# Autodesk Inventor assembly: Zusammenbau
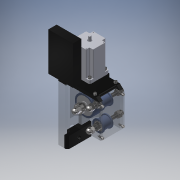
[picture p0: Inventor's stored thumbnail of the model, 180x180]
Saved by Autodesk Inventor 2019 (Build 230136000, 136)
## iProperties
Created: 2021-11-05
Part Number: Zusammenbau
Material: Generisch
Document SubType Name: Assembly
Designer: Bergi
Author: Bergi
## Documents named in this file (26)
- C:\Users\Bergi\Desktop\3D Sketches\Jalousie_Motor\Zusammenbau.iam
- C:\Users\Bergi\Desktop\3D Sketches\Jalousie_Motor\Nema23(SY60STH86-3008).ipt
- C:\Users\Bergi\Desktop\3D Sketches\Jalousie_Motor\Schneckenrad.ipt
- C:\Users\Bergi\Desktop\3D Sketches\Jalousie_Motor\Schneckenwelle.ipt
- C:\Users\Bergi\Desktop\3D Sketches\Jalousie_Motor\Gummiwalze.ipt
- C:\Users\Bergi\Desktop\3D Sketches\Jalousie_Motor\ABS Walze.ipt
- C:\Users\Bergi\Desktop\3D Sketches\Jalousie_Motor\DIN 625 T1 - 6000 - 10 x 26 x 8.ipt
- C:\Users\Bergi\Desktop\3D Sketches\Jalousie_Motor\Gewindestange.ipt
- C:\Users\Bergi\Desktop\3D Sketches\Jalousie_Motor\DIN 934 - M10 x 1,5.ipt
- C:\Users\Bergi\Desktop\3D Sketches\Jalousie_Motor\DIN 988 - 10 x 16 x 1.ipt
- C:\Users\Bergi\Desktop\3D Sketches\Jalousie_Motor\Frame.ipt
- C:\Users\Bergi\Desktop\3D Sketches\Jalousie_Motor\DIN 1587 - M10 x 1,25.ipt
- C:\Users\Bergi\Desktop\3D Sketches\Jalousie_Motor\Shaft Kupplung.ipt
- C:\Users\Bergi\Desktop\3D Sketches\Jalousie_Motor\Deckel_Frame.ipt
- C:\Users\Bergi\Desktop\3D Sketches\Jalousie_Motor\DIN 625 T1 - 626 - 6 x 19 x 6.ipt
- C:\Users\Bergi\Desktop\3D Sketches\Jalousie_Motor\Holding_Plate_Frame.ipt
- C:\Users\Bergi\Desktop\3D Sketches\Jalousie_Motor\Deckel_2_Frame.ipt
- C:\Users\Bergi\Desktop\3D Sketches\Jalousie_Motor\DIN 912 - M4 x 0,7 x 10 x 8,25.ipt
- C:\Users\Bergi\Desktop\3D Sketches\Jalousie_Motor\DIN 912 - M5 x 0,8 x 16 x 14.ipt
- C:\Users\Bergi\Desktop\3D Sketches\Jalousie_Motor\Stepperdriver.ipt
- C:\Users\Bergi\Desktop\3D Sketches\Jalousie_Motor\Zusammenbau\AIP\FEA\ds3uq4s4g.fins
- C:\Users\Bergi\Desktop\3D Sketches\Jalousie_Motor\Zusammenbau\AIP\FEA\ds3uq4s4g.fsat
- C:\Users\Bergi\Desktop\3D Sketches\Jalousie_Motor\Zusammenbau\AIP\FEA\ds3uq4s4g.ftes
- C:\Users\Bergi\Desktop\3D Sketches\Jalousie_Motor\Zusammenbau\AIP\FEA\ds3uq4s5c.fwiz
- C:\Users\Bergi\Desktop\3D Sketches\Jalousie_Motor\Zusammenbau\AIP\FEA\ds3uq4sdc.fmsh
- C:\Users\Bergi\Desktop\3D Sketches\Jalousie_Motor\Zusammenbau\AIP\FEA\ds3uq4sdd.fres
## Components (51 placed, 19 different names)
1. Nema23(SY60STH86-3008):1 — Passend:1, Winkel:1, Winkel:3, Passend:68, Winkel:4, Passend:69, Passend:71, Passend:92, Passend:93, Passend:94, Passend:95, Passend:96, Passend:97, Passend:98, Passend:99, Fluchtend:8
2. Schneckenrad:1 — Passend:2, Passend:3, Winkel:1, Passend:4, Passend:13, Passend:18
3. Schneckenwelle:1 — Passend:1, Passend:2, Passend:3
4. Gummiwalze:1 — Passend:4, Passend:13, Passend:14, Passend:16, Fluchtend:1, Passend:31
5. ABS Walze:1 — Passend:5, Passend:6, Passend:7, Passend:8, Fluchtend:1
6. DIN 625 - T1 6000 - 10 x 26 x 8:1 — Passend:6, Passend:7, Passend:36
7. DIN 625 - T1 6000 - 10 x 26 x 8:2 — Passend:5, Passend:8, Winkel:2, Passend:32, Passend:34
8. ABS Walze:2 — Passend:31
9. DIN 625 - T1 6000 - 10 x 26 x 8:3 — Passend:37, Passend:41
10. DIN 625 - T1 6000 - 10 x 26 x 8:4 — Passend:40
11. Gewindestange:1 — Passend:14, Passend:15, Passend:17, Passend:19, Passend:21, Passend:23, Passend:25, Winkel:2, Fluchtend:2, Fluchtend:3, Passend:52, Passend:54
12. DIN 934 - ersetzt durch DIN EN 24032/28673/28674 M10:1 — Passend:19, Passend:20, Passend:22
13. DIN 988 10 x 16 x 1:1 — Passend:15, Passend:16, Passend:24
14. DIN 988 10 x 16 x 1:2 — Passend:17, Passend:18, Passend:20
15. DIN 625 - T1 6000 - 10 x 26 x 8:5 — Passend:21, Passend:22, Passend:55
16. DIN 934 - ersetzt durch DIN EN 24032/28673/28674 M10:2 — Passend:23, Passend:24, Passend:26
17. DIN 625 - T1 6000 - 10 x 26 x 8:6 — Passend:25, Passend:26, Passend:42, Passend:43, Passend:53
18. Gewindestange:2 — Passend:32, Passend:33, Passend:35, Fluchtend:2, Passend:44, Passend:47, Passend:50, Passend:56, Passend:58
19. DIN 934 - ersetzt durch DIN EN 24032/28673/28674 M10:5 — Passend:33, Passend:34
20. DIN 934 - ersetzt durch DIN EN 24032/28673/28674 M10:6 — Passend:35, Passend:36
21. Gewindestange:3 — Passend:37, Passend:38, Passend:39, Fluchtend:3, Passend:45, Fluchtend:4, Passend:60, Passend:62, Passend:64, Passend:66
22. DIN 934 - ersetzt durch DIN EN 24032/28673/28674 M10:7 — Passend:38, Passend:41
23. DIN 934 - ersetzt durch DIN EN 24032/28673/28674 M10:8 — Passend:39, Passend:40
24. Frame:1 — Passend:42, Passend:43, Winkel:3, Passend:44, Passend:45, Passend:48, Passend:51, Fluchtend:4, Passend:61, Passend:63, Passend:70, Fluchtend:5, Fluchtend:6, Passend:72, Passend:73, Passend:74, Passend:75, Fluchtend:7, Passend:77, Passend:78, Passend:79
25. DIN 988 10 x 16 x 1:3 — Passend:47, Passend:48, Passend:57
26. DIN 988 10 x 16 x 1:4 — Passend:50, Passend:51, Passend:59
27. DIN 1587 M10 x 1,25 - SW16:1 — Passend:52, Passend:53
28. DIN 1587 M10 x 1,25 - SW16:2 — Passend:54, Passend:55
29. DIN 1587 M10 x 1,25 - SW16:3 — Passend:56, Passend:57
30. DIN 1587 M10 x 1,25 - SW16:4 — Passend:58, Passend:59
31. DIN 988 10 x 16 x 1:5 — Passend:60, Passend:61, Passend:67
32. DIN 988 10 x 16 x 1:6 — Passend:62, Passend:63, Passend:65
33. DIN 1587 M10 x 1,25 - SW16:5 — Passend:64, Passend:65
34. DIN 1587 M10 x 1,25 - SW16:6 — Passend:66, Passend:67
35. Shaft Kupplung:1 — Passend:68, Winkel:4, Passend:69, Passend:76
36. Deckel_Frame:1 — Passend:70, Fluchtend:5, Fluchtend:6, Passend:71, Passend:76, Passend:88, Passend:89, Passend:90, Passend:91, Passend:100, Passend:101
37. DIN 625 - T1 626 - 6 x 19 x 6:1 — Passend:72, Passend:73
38. Holding_Plate_Frame:1 — Passend:74, Passend:75, Fluchtend:7
39. Deckel_2_Frame:1 — Passend:77, Passend:78, Passend:79, Passend:80, Passend:81, Passend:82, Passend:83, Passend:84, Passend:85, Passend:86, Passend:87
40. DIN 912 - ersetzt durch DIN EN ISO 4762 M4 x 10:1 — Passend:80, Passend:81
41. DIN 912 - ersetzt durch DIN EN ISO 4762 M4 x 10:2 — Passend:82, Passend:83
42. DIN 912 - ersetzt durch DIN EN ISO 4762 M4 x 10:3 — Passend:84, Passend:85
43. DIN 912 - ersetzt durch DIN EN ISO 4762 M4 x 10:4 — Passend:86, Passend:87
44. DIN 912 - ersetzt durch DIN EN ISO 4762 M5 x 16:1 — Passend:88, Passend:89
45. DIN 912 - ersetzt durch DIN EN ISO 4762 M5 x 16:2 — Passend:90, Passend:91
46. DIN 912 - ersetzt durch DIN EN ISO 4762 M5 x 16:3 — Passend:92, Passend:98
47. DIN 912 - ersetzt durch DIN EN ISO 4762 M5 x 16:4 — Passend:95, Passend:96
48. DIN 912 - ersetzt durch DIN EN ISO 4762 M5 x 16:5 — Passend:94, Passend:99
49. DIN 912 - ersetzt durch DIN EN ISO 4762 M5 x 16:6 — Passend:93, Passend:97
50. DIN 912 - ersetzt durch DIN EN ISO 4762 M5 x 16:7 — Passend:100, Passend:101
51. Stepperdriver:1 — Fluchtend:8
## Relationships (107: Mate 95, Flush 8, Angle 4)
- Passend:1 [Mate]: Nema23(SY60STH86-3008):1 ↔ Schneckenwelle:1
- Passend:2 [Mate]: Schneckenrad:1 ↔ Schneckenwelle:1
- Passend:3 [Mate] (-6.5 mm): Schneckenrad:1 ↔ Schneckenwelle:1
- Winkel:1 [Angle] (-90 deg): Nema23(SY60STH86-3008):1 ↔ Schneckenrad:1
- Passend:4 [Mate]: Schneckenrad:1 ↔ Gummiwalze:1
- Passend:5 [Mate]: ABS Walze:1 ↔ DIN 625 - T1 6000 - 10 x 26 x 8:2
- Passend:6 [Mate]: ABS Walze:1 ↔ DIN 625 - T1 6000 - 10 x 26 x 8:1
- Passend:7 [Mate]: ABS Walze:1 ↔ DIN 625 - T1 6000 - 10 x 26 x 8:1
- Passend:8 [Mate]: ABS Walze:1 ↔ DIN 625 - T1 6000 - 10 x 26 x 8:2
- [Mate]: ABS Walze:2 ↔ DIN 625 - T1 6000 - 10 x 26 x 8:4
- [Mate]: ABS Walze:2 ↔ DIN 625 - T1 6000 - 10 x 26 x 8:3
- [Mate]: ABS Walze:2 ↔ DIN 625 - T1 6000 - 10 x 26 x 8:3
- [Mate]: ABS Walze:2 ↔ DIN 625 - T1 6000 - 10 x 26 x 8:4
- Passend:13 [Mate]: Schneckenrad:1 ↔ Gummiwalze:1
- Passend:14 [Mate]: Gummiwalze:1 ↔ Gewindestange:1
- Passend:15 [Mate]: Gewindestange:1 ↔ DIN 988 10 x 16 x 1:1
- Passend:16 [Mate]: Gummiwalze:1 ↔ DIN 988 10 x 16 x 1:1
- Passend:17 [Mate]: Gewindestange:1 ↔ DIN 988 10 x 16 x 1:2
- Passend:18 [Mate]: Schneckenrad:1 ↔ DIN 988 10 x 16 x 1:2
- Passend:19 [Mate]: Gewindestange:1 ↔ DIN 934 - ersetzt durch DIN EN 24032/28673/28674 M10:1
- Passend:20 [Mate]: DIN 934 - ersetzt durch DIN EN 24032/28673/28674 M10:1 ↔ DIN 988 10 x 16 x 1:2
- Passend:21 [Mate]: Gewindestange:1 ↔ DIN 625 - T1 6000 - 10 x 26 x 8:5
- Passend:22 [Mate]: DIN 934 - ersetzt durch DIN EN 24032/28673/28674 M10:1 ↔ DIN 625 - T1 6000 - 10 x 26 x 8:5
- Passend:23 [Mate]: Gewindestange:1 ↔ DIN 934 - ersetzt durch DIN EN 24032/28673/28674 M10:2
- Passend:24 [Mate]: DIN 988 10 x 16 x 1:1 ↔ DIN 934 - ersetzt durch DIN EN 24032/28673/28674 M10:2
- Passend:25 [Mate]: Gewindestange:1 ↔ DIN 625 - T1 6000 - 10 x 26 x 8:6
- Passend:26 [Mate]: DIN 934 - ersetzt durch DIN EN 24032/28673/28674 M10:2 ↔ DIN 625 - T1 6000 - 10 x 26 x 8:6
- Winkel:2 [Angle] (0 deg): DIN 625 - T1 6000 - 10 x 26 x 8:2 ↔ Gewindestange:1
- Fluchtend:1 [Flush]: Gummiwalze:1 ↔ ABS Walze:1
- Passend:31 [Mate]: Gummiwalze:1 ↔ ABS Walze:2
- Passend:32 [Mate]: DIN 625 - T1 6000 - 10 x 26 x 8:2 ↔ Gewindestange:2
- Passend:33 [Mate]: Gewindestange:2 ↔ DIN 934 - ersetzt durch DIN EN 24032/28673/28674 M10:5
- Passend:34 [Mate]: DIN 625 - T1 6000 - 10 x 26 x 8:2 ↔ DIN 934 - ersetzt durch DIN EN 24032/28673/28674 M10:5
- Passend:35 [Mate]: Gewindestange:2 ↔ DIN 934 - ersetzt durch DIN EN 24032/28673/28674 M10:6
- Passend:36 [Mate]: DIN 625 - T1 6000 - 10 x 26 x 8:1 ↔ DIN 934 - ersetzt durch DIN EN 24032/28673/28674 M10:6
- Passend:37 [Mate]: DIN 625 - T1 6000 - 10 x 26 x 8:3 ↔ Gewindestange:3
- Passend:38 [Mate]: Gewindestange:3 ↔ DIN 934 - ersetzt durch DIN EN 24032/28673/28674 M10:7
- Passend:39 [Mate]: Gewindestange:3 ↔ DIN 934 - ersetzt durch DIN EN 24032/28673/28674 M10:8
- Passend:40 [Mate]: DIN 625 - T1 6000 - 10 x 26 x 8:4 ↔ DIN 934 - ersetzt durch DIN EN 24032/28673/28674 M10:8
- Passend:41 [Mate]: DIN 625 - T1 6000 - 10 x 26 x 8:3 ↔ DIN 934 - ersetzt durch DIN EN 24032/28673/28674 M10:7
- Fluchtend:2 [Flush]: Gewindestange:1 ↔ Gewindestange:2
- Fluchtend:3 [Flush]: Gewindestange:1 ↔ Gewindestange:3
- Passend:42 [Mate]: DIN 625 - T1 6000 - 10 x 26 x 8:6 ↔ Frame:1
- Passend:43 [Mate]: DIN 625 - T1 6000 - 10 x 26 x 8:6 ↔ Frame:1
- Winkel:3 [Angle] (0 deg): Nema23(SY60STH86-3008):1 ↔ Frame:1
- Passend:44 [Mate]: Gewindestange:2 ↔ Frame:1
- Passend:45 [Mate]: Gewindestange:3 ↔ Frame:1
- Passend:47 [Mate]: Gewindestange:2 ↔ DIN 988 10 x 16 x 1:3
- Passend:48 [Mate]: Frame:1 ↔ DIN 988 10 x 16 x 1:3
- Passend:50 [Mate]: Gewindestange:2 ↔ DIN 988 10 x 16 x 1:4
- Passend:51 [Mate]: Frame:1 ↔ DIN 988 10 x 16 x 1:4
- Passend:52 [Mate]: Gewindestange:1 ↔ DIN 1587 M10 x 1,25 - SW16:1
- Passend:53 [Mate]: DIN 625 - T1 6000 - 10 x 26 x 8:6 ↔ DIN 1587 M10 x 1,25 - SW16:1
- Passend:54 [Mate]: Gewindestange:1 ↔ DIN 1587 M10 x 1,25 - SW16:2
- Passend:55 [Mate]: DIN 625 - T1 6000 - 10 x 26 x 8:5 ↔ DIN 1587 M10 x 1,25 - SW16:2
- Passend:56 [Mate]: Gewindestange:2 ↔ DIN 1587 M10 x 1,25 - SW16:3
- Passend:57 [Mate]: DIN 988 10 x 16 x 1:3 ↔ DIN 1587 M10 x 1,25 - SW16:3
- Passend:58 [Mate]: Gewindestange:2 ↔ DIN 1587 M10 x 1,25 - SW16:4
- Passend:59 [Mate]: DIN 988 10 x 16 x 1:4 ↔ DIN 1587 M10 x 1,25 - SW16:4
- Fluchtend:4 [Flush] (8 mm): Gewindestange:3 ↔ Frame:1
- Passend:60 [Mate]: Gewindestange:3 ↔ DIN 988 10 x 16 x 1:5
- Passend:61 [Mate]: Frame:1 ↔ DIN 988 10 x 16 x 1:5
- Passend:62 [Mate]: Gewindestange:3 ↔ DIN 988 10 x 16 x 1:6
- Passend:63 [Mate]: Frame:1 ↔ DIN 988 10 x 16 x 1:6
- Passend:64 [Mate]: Gewindestange:3 ↔ DIN 1587 M10 x 1,25 - SW16:5
- Passend:65 [Mate]: DIN 988 10 x 16 x 1:6 ↔ DIN 1587 M10 x 1,25 - SW16:5
- Passend:66 [Mate]: Gewindestange:3 ↔ DIN 1587 M10 x 1,25 - SW16:6
- Passend:67 [Mate]: DIN 988 10 x 16 x 1:5 ↔ DIN 1587 M10 x 1,25 - SW16:6
- Passend:68 [Mate]: Nema23(SY60STH86-3008):1 ↔ Shaft Kupplung:1
- Winkel:4 [Angle] (0 deg): Nema23(SY60STH86-3008):1 ↔ Shaft Kupplung:1
- Passend:69 [Mate] (1 mm): Nema23(SY60STH86-3008):1 ↔ Shaft Kupplung:1
- Passend:70 [Mate]: Frame:1 ↔ Deckel_Frame:1
- Fluchtend:5 [Flush]: Frame:1 ↔ Deckel_Frame:1
- Fluchtend:6 [Flush]: Frame:1 ↔ Deckel_Frame:1
- Passend:71 [Mate]: Nema23(SY60STH86-3008):1 ↔ Deckel_Frame:1
- Passend:72 [Mate]: Frame:1 ↔ DIN 625 - T1 626 - 6 x 19 x 6:1
- Passend:73 [Mate]: Frame:1 ↔ DIN 625 - T1 626 - 6 x 19 x 6:1
- Passend:74 [Mate]: Frame:1 ↔ Holding_Plate_Frame:1
- Passend:75 [Mate]: Frame:1 ↔ Holding_Plate_Frame:1
- Fluchtend:7 [Flush]: Frame:1 ↔ Holding_Plate_Frame:1
- Passend:76 [Mate]: Shaft Kupplung:1 ↔ Deckel_Frame:1
- Passend:77 [Mate]: Frame:1 ↔ Deckel_2_Frame:1
- Passend:78 [Mate]: Frame:1 ↔ Deckel_2_Frame:1
- Passend:79 [Mate]: Frame:1 ↔ Deckel_2_Frame:1
- Passend:80 [Mate]: Deckel_2_Frame:1 ↔ DIN 912 - ersetzt durch DIN EN ISO 4762 M4 x 10:1
- Passend:81 [Mate]: Deckel_2_Frame:1 ↔ DIN 912 - ersetzt durch DIN EN ISO 4762 M4 x 10:1
- Passend:82 [Mate]: Deckel_2_Frame:1 ↔ DIN 912 - ersetzt durch DIN EN ISO 4762 M4 x 10:2
- Passend:83 [Mate]: Deckel_2_Frame:1 ↔ DIN 912 - ersetzt durch DIN EN ISO 4762 M4 x 10:2
- Passend:84 [Mate]: Deckel_2_Frame:1 ↔ DIN 912 - ersetzt durch DIN EN ISO 4762 M4 x 10:3
- Passend:85 [Mate]: Deckel_2_Frame:1 ↔ DIN 912 - ersetzt durch DIN EN ISO 4762 M4 x 10:3
- Passend:86 [Mate]: Deckel_2_Frame:1 ↔ DIN 912 - ersetzt durch DIN EN ISO 4762 M4 x 10:4
- Passend:87 [Mate]: Deckel_2_Frame:1 ↔ DIN 912 - ersetzt durch DIN EN ISO 4762 M4 x 10:4
- Passend:88 [Mate]: Deckel_Frame:1 ↔ DIN 912 - ersetzt durch DIN EN ISO 4762 M5 x 16:1
- Passend:89 [Mate]: Deckel_Frame:1 ↔ DIN 912 - ersetzt durch DIN EN ISO 4762 M5 x 16:1
- Passend:90 [Mate]: Deckel_Frame:1 ↔ DIN 912 - ersetzt durch DIN EN ISO 4762 M5 x 16:2
- Passend:91 [Mate]: Deckel_Frame:1 ↔ DIN 912 - ersetzt durch DIN EN ISO 4762 M5 x 16:2
- Passend:92 [Mate]: Nema23(SY60STH86-3008):1 ↔ DIN 912 - ersetzt durch DIN EN ISO 4762 M5 x 16:3
- Passend:93 [Mate]: Nema23(SY60STH86-3008):1 ↔ DIN 912 - ersetzt durch DIN EN ISO 4762 M5 x 16:6
- Passend:94 [Mate]: Nema23(SY60STH86-3008):1 ↔ DIN 912 - ersetzt durch DIN EN ISO 4762 M5 x 16:5
- Passend:95 [Mate]: Nema23(SY60STH86-3008):1 ↔ DIN 912 - ersetzt durch DIN EN ISO 4762 M5 x 16:4
- Passend:96 [Mate]: Nema23(SY60STH86-3008):1 ↔ DIN 912 - ersetzt durch DIN EN ISO 4762 M5 x 16:4
- Passend:97 [Mate]: Nema23(SY60STH86-3008):1 ↔ DIN 912 - ersetzt durch DIN EN ISO 4762 M5 x 16:6
- Passend:98 [Mate]: Nema23(SY60STH86-3008):1 ↔ DIN 912 - ersetzt durch DIN EN ISO 4762 M5 x 16:3
- Passend:99 [Mate]: Nema23(SY60STH86-3008):1 ↔ DIN 912 - ersetzt durch DIN EN ISO 4762 M5 x 16:5
- Passend:100 [Mate]: Deckel_Frame:1 ↔ DIN 912 - ersetzt durch DIN EN ISO 4762 M5 x 16:7
- Passend:101 [Mate]: Deckel_Frame:1 ↔ DIN 912 - ersetzt durch DIN EN ISO 4762 M5 x 16:7
- Fluchtend:8 [Flush]: Nema23(SY60STH86-3008):1 ↔ Stepperdriver:1
## Named parameters: d9_d5 = 0 mm, d10_d6 = 0 mm, d11_d7 = 0 mm, d12_d8 = 0 mm, sa_0 = 37.5
note: some values were not read from the file. Shown as the stored number, unit unknown: "sa_0".
